# Autodesk Inventor assembly: 针头主体
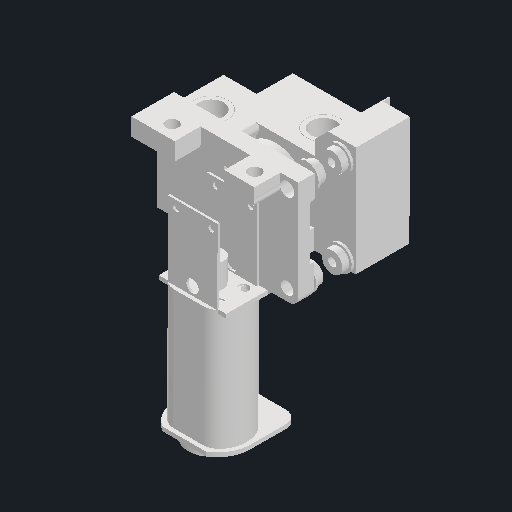
[picture p0: Inventor's stored thumbnail of the model, 512x512]
Saved by Autodesk Inventor 2025 (Build 290162000, 162)
## iProperties
Created: 2025-12-02
Part Number: 针头主体
Document SubType Name: Assembly
Designer: XH
Author: XH
## Documents named in this file (8)
- C:\1A_Engineering_files\braille-printer-v2\3D文件\针头主体.iam
- C:\1A_Engineering_files\braille-printer-v2\3D文件\电机.ipt
- C:\1A_Engineering_files\braille-printer-v2\3D文件\电机装配.ipt
- C:\1A_Engineering_files\braille-printer-v2\3D文件\皮带轮.ipt
- C:\1A_Engineering_files\braille-printer-v2\3D文件\固定传动.ipt
- C:\1A_Engineering_files\braille-printer-v2\3D文件\小轴承.ipt
- C:\1A_Engineering_files\braille-printer-v2\3D文件\铜套.ipt
- C:\1A_Engineering_files\braille-printer-v2\3D文件\MPU 6050 IMU.iam
## Components (13 placed, 7 different names)
1. 电机:1 — 配合:10, 配合:14
2. 电机装配:1 — 配合:10, 配合:16, 表面齐平:1
3. 皮带轮:1 — 配合:14
4. 固定传动:1 — 配合:16, 表面齐平:1, 配合:21, 表面齐平:5, 配合:22, 表面齐平:6, 配合:23, 表面齐平:7, 配合:24, 表面齐平:8, 配合:25, 配合:26, 配合:27
5. 小轴承:1 — 配合:18, 表面齐平:3, 配合:27
6. 小轴承:2 — 配合:18, 表面齐平:4
7. 小轴承:3 — 表面齐平:3
8. 小轴承:4 — 表面齐平:4
9. 铜套:1 — 配合:21, 表面齐平:5
10. 铜套:2 — 配合:22, 表面齐平:6
11. 铜套:3 — 配合:23, 表面齐平:7
12. 铜套:4 — 配合:24, 表面齐平:8
13. MPU 6050 IMU:1 [sub-assembly] — 配合:25, 配合:26
## Relationships (19: Mate 12, Flush 7)
- 配合:10 [Mate]: 电机:1 ↔ 电机装配:1
- 配合:14 [Mate]: 电机:1 ↔ 皮带轮:1
- 配合:16 [Mate]: 电机装配:1 ↔ 固定传动:1
- 表面齐平:1 [Flush]: 电机装配:1 ↔ 固定传动:1
- 配合:18 [Mate]: 小轴承:1 ↔ 小轴承:2
- [Mate]: 小轴承:3 ↔ 小轴承:4
- 表面齐平:3 [Flush]: 小轴承:1 ↔ 小轴承:3
- 表面齐平:4 [Flush]: 小轴承:2 ↔ 小轴承:4
- 配合:21 [Mate]: 固定传动:1 ↔ 铜套:1
- 表面齐平:5 [Flush]: 固定传动:1 ↔ 铜套:1
- 配合:22 [Mate]: 固定传动:1 ↔ 铜套:2
- 表面齐平:6 [Flush]: 固定传动:1 ↔ 铜套:2
- 配合:23 [Mate]: 固定传动:1 ↔ 铜套:3
- 表面齐平:7 [Flush]: 固定传动:1 ↔ 铜套:3
- 配合:24 [Mate]: 固定传动:1 ↔ 铜套:4
- 表面齐平:8 [Flush]: 固定传动:1 ↔ 铜套:4
- 配合:25 [Mate]: 固定传动:1 ↔ MPU 6050 IMU:1
- 配合:26 [Mate]: 固定传动:1 ↔ MPU 6050 IMU:1
- 配合:27 [Mate]: 固定传动:1 ↔ 小轴承:1
## Named parameters: d25_d23 = 0 mm
